# Autodesk Inventor assembly: PWTR-0033
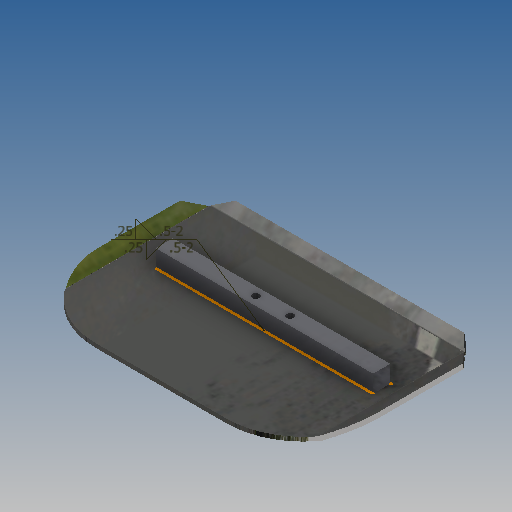
[picture p0: Inventor's stored thumbnail of the model, 512x512]
Saved by Autodesk Inventor 2021.1 (Build 251245000, 245)
## iProperties
Part Number: PWTR-0033
Document SubType Name: Weldment
Created: 2003-02-05
Designer: B. BOGAN
Description: TROWEL WELDMENT
Weld Material: Welded Aluminum-6061
Vendor: Design Specific
Control State: 0
Master: False
Checked Out: False
Shininess: 64.0
Length Units: 11272
Angle Units: 11279
Time Units: 11290
Mass Units: 11286
Length Display Precision: 3
Angle Display Precision: 2
Compacted: True
Density: 0.0
Volumn: 0.0
Area: 0.0
PropertySet Name: Model Information
Title: TROWEL WELDMENT
Author: B. BOGAN
Revision Number: B
## Documents named in this file (3)
- C:\Vault Workspace\Design Data\Projects\PRJ0095\PWTR-Components\PWTR-0033.iam
- C:\Vault Workspace\Design Data\Projects\PRJ0095\PWTR-Components\PWTR-0042.ipt
- C:\Vault Workspace\Design Data\Projects\PRJ0095\PWTR-Components\PWTR-0041.ipt
## Components (2 placed, 2 different names)
1. TROWEL — Mate:1, Mate:2, Flush:1
2. TROWEL SUPPORT — Mate:1, Mate:2, Flush:1
## Relationships (3: Mate 2, Flush 1)
- Mate:1: TROWEL ↔ TROWEL SUPPORT
- Mate:2 (19.05 mm): TROWEL ↔ TROWEL SUPPORT
- Flush:1 (-69.85 mm): TROWEL ↔ TROWEL SUPPORT
